# Autodesk Inventor assembly: Assembly1
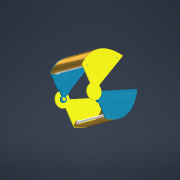
[picture p0: Inventor's stored thumbnail of the model, 180x180]
Saved by Autodesk Inventor 2021 (Build 250183000, 183)
## iProperties
Created: 2021-02-13
Part Number: Assembly1
Document SubType Name: Assembly
Designer: vikki
Mass: 64.2382 g
Surface Area: 532.982 cm^2
Volume: 60.6021 cm^3
Density: 1.06 g/cm^3
Author: vikki
## Documents named in this file (5)
- D:\borewell rescuebot\pll manipulator files\sps manipulator\Assembly1.iam
- D:\borewell rescuebot\pll manipulator files\sps manipulator\clamshell half.ipt
- D:\borewell rescuebot\pll manipulator files\sps manipulator\clamshell half-2.ipt
- D:\borewell rescuebot\pll manipulator files\sps manipulator\clamshell cross link.ipt
- D:\borewell rescuebot\pll manipulator files\sps manipulator\clamsheel sheet surface.ipt
## Components (10 placed, 4 different names)
1. clamshell half:3
2. clamshell half-2:3
3. clamshell half:4
4. clamshell half-2:4
5. clamshell cross link:5
6. clamshell cross link:6
7. clamshell cross link:7
8. clamshell cross link:8
9. clamsheel sheet surface:1
10. clamsheel sheet surface:2
## Relationships (20: Mate 11, Flush 9)
- [Flush]: clamshell half:3 ↔ clamshell half-2:3
- [Mate]: clamshell half:3 ↔ clamshell half-2:3
- [Mate]: clamshell half:4 ↔ clamshell half-2:4
- [Flush]: clamshell half:4 ↔ clamshell half-2:4
- [Flush]: clamshell half-2:3 ↔ clamshell half:4
- [Flush]: clamshell half:3 ↔ clamshell half-2:4
- [Mate]: clamshell half:3 ↔ clamshell cross link:5
- [Mate]: clamshell half:3 ↔ clamshell cross link:6
- [Mate]: clamshell half-2:3 ↔ clamshell cross link:7
- [Mate]: clamshell half-2:3 ↔ clamshell cross link:7
- [Mate]: clamshell half-2:3 ↔ clamshell cross link:8
- [Mate]: clamshell half-2:3 ↔ clamshell cross link:8
- [Mate]: clamshell half-2:4 ↔ clamshell cross link:5
- [Mate]: clamshell half-2:4 ↔ clamshell cross link:6
- [Flush]: clamshell half-2:3 ↔ clamsheel sheet surface:1
- [Mate]: clamshell half:3 ↔ clamsheel sheet surface:2
- [Flush]: clamshell half:3 ↔ clamsheel sheet surface:2
- [Flush]: clamshell half:3 ↔ clamsheel sheet surface:2
- [Flush]: clamshell half:4 ↔ clamsheel sheet surface:1
- [Flush]: clamshell half:4 ↔ clamsheel sheet surface:1
## Named parameters: d27_d303 = 0 mm, d28_d304 = 0 mm, d29_d305 = 0 mm, d30_d307 = 0 mm, d31_d309 = 0 mm, d32_d289 = 0 mm, d33_d291 = 0 mm, d34_d302 = 0 mm, d35_d310 = 0 mm, d36_d311 = 0 mm, d37_d312 = 0 mm, d38_d313 = 0 mm
